# Autodesk Inventor assembly: Futaba_RS30x
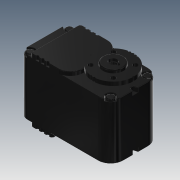
[picture p0: Inventor's stored thumbnail of the model, 180x180]
Saved by Autodesk Inventor 2018 (Build 220112000, 112)
## iProperties
Created: 2018-05-24
Part Number: Futaba_RS30x
Material: 一般
Document SubType Name: Assembly
Designer: y6tada
Author: y6tada
## Documents named in this file (3)
- C:\Users\y6tada\Dropbox\曹研究室\多田\Intel NUC Hexapod\Inventor\Futaba_RS30x\Futaba_RS30x.iam
- C:\Users\y6tada\Dropbox\曹研究室\多田\Intel NUC Hexapod\Inventor\Futaba_RS30x\RS30x.ipt
- C:\Users\y6tada\Dropbox\曹研究室\多田\Intel NUC Hexapod\Inventor\Futaba_RS30x\RS30x_ServoHorn.ipt
## Components (2 placed, 2 different names)
1. RS30x:1 — メイト:1, メイト:2
2. RS30x_ServoHorn:1 — メイト:1, メイト:2, 角度:1
## Relationships (3: Mate 2, Angle 1)
- メイト:1 [Mate]: RS30x:1 ↔ RS30x_ServoHorn:1
- メイト:2 [Mate]: RS30x:1 ↔ RS30x_ServoHorn:1
- 角度:1 [Angle] (180 deg): RS30x_ServoHorn:1
